# Autodesk Inventor assembly: maze_version2
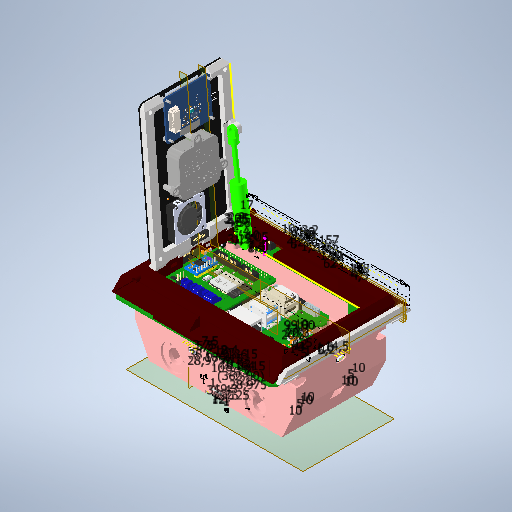
[picture p0: Inventor's stored thumbnail of the model, 512x512]
Saved by Autodesk Inventor 2025 (Build 290162000, 162)
## iProperties
Created: 2026-06-23
Part Number: maze_version2
Document SubType Name: Assembly
Designer: garin
Author: garin
## Documents named in this file (20)
- C:\Users\Leva\Documents\Git\TheseusV2_Maze\Construction\Theseus_v2\Theseus_v2.iam
- C:\Users\Leva\Documents\Git\TheseusV2_Maze\Construction\Theseus_v2\DDSM210.ipt
- C:\Users\Leva\Documents\Git\TheseusV2_Maze\Construction\akkum_TSE\akkum.iam
- C:\Users\Leva\Documents\Git\TheseusV2_Maze\Construction\Theseus_v2\low_part.ipt
- C:\Users\Leva\Documents\Git\TheseusV2_Maze\Construction\Theseus_v2\USBCamera.ipt
- C:\Users\Leva\Documents\Git\TheseusV2_Maze\Construction\maze_test_course\maze_test_course.ipt
- C:\Users\Leva\Documents\Git\TheseusV2_Maze\Construction\Theseus_v2\TCS34725.ipt
- C:\Users\Leva\Documents\Git\TheseusV2_Maze\Construction\Theseus_v2\optopar.ipt
- C:\Users\Leva\Documents\Git\TheseusV2_Maze\Construction\Theseus_v2\magasin.ipt
- C:\Users\Leva\Documents\Git\TheseusV2_Maze\Construction\Theseus_v2\mother_board\mb_mother_board.iam
- C:\Users\Leva\Documents\Git\TheseusV2_Maze\Construction\Theseus_v2\OCS-D008 B.ipt
- C:\Users\Leva\Documents\Git\TheseusV2_Maze\Construction\Theseus_v2\up_part.ipt
- C:\Users\Leva\Documents\Git\TheseusV2_Maze\Construction\Theseus_v2\microswitch_cap.ipt
- C:\Users\Leva\Documents\Git\TheseusV2_Maze\Construction\Theseus_v2\microswitch_cap_MIR.ipt
- C:\Users\Leva\Documents\Git\TheseusV2_Maze\Schematic\TSE_power_control_board\model\TSE_power_control_board.iam
- C:\Users\Leva\Documents\Git\TheseusV2_Maze\Schematic\TSE_sensor_commutation_board\model\TSE_sensor_commutation_board.iam
- C:\Users\Leva\Documents\Git\TheseusV2_Maze\Schematic\TSE_commutation_board\model\TSE_commutation_board.iam
- C:\Users\Leva\Documents\Git\TheseusV2_Maze\Construction\Theseus_v2\cap.ipt
- C:\Users\Leva\Documents\Git\TheseusV2_Maze\Construction\Theseus_v2\gaslift_YQ4-12_body.ipt
- C:\Users\Leva\Documents\Git\TheseusV2_Maze\Construction\Theseus_v2\gaslift_YQ4-12_rod.ipt
## Components (26 placed, 19 different names)
1. low_part:1 — Заподлицо:1, Заподлицо:2, Заподлицо:3, Совмещение:1, Совмещение:2, Совмещение:3, Совмещение:7, Совмещение:8, Совмещение:9, Совмещение:27, Совмещение:28, Совмещение:29, Совмещение:30, Совмещение:31, Совмещение:32, Совмещение:42, Совмещение:43, Совмещение:44, Совмещение:45, Совмещение:46, Совмещение:47, Совмещение:49, Угол:1, Совмещение:62, Совмещение:63, Заподлицо:14, Совмещение:64, Совмещение:65, Заподлицо:18, Совмещение:68, Совмещение:122, Заподлицо:117, Совмещение:123, Совмещение:124, Совмещение:125, Совмещение:129, Заподлицо:118, Заподлицо:119, Заподлицо:122
2. DDSM210:1 — Совмещение:27, Совмещение:28, Совмещение:29, Заподлицо:19
3. DDSM210:2 — Совмещение:1, Совмещение:2, Совмещение:3
4. DDSM210:3 — Совмещение:30, Совмещение:31, Совмещение:32
5. DDSM210:4 — Совмещение:7, Совмещение:8, Совмещение:9
6. akkum:2 [sub-assembly] — Совмещение:122, Заподлицо:117
7. maze_test_course:1 — Совмещение:35
8. TCS34725:1 — Совмещение:45, Совмещение:46, Совмещение:47
9. optopar:1 — Совмещение:42, Совмещение:43, Совмещение:44
10. USBCamera:2 — Совмещение:49, Угол:1, Совмещение:68
11. magasin:1 — Совмещение:62, Совмещение:63, Заподлицо:14, Заподлицо:15
12. mb_mother_board:1 [sub-assembly] — Совмещение:126, Совмещение:127, Совмещение:128
13. OCS-D008 B:1 — Заподлицо:15, Совмещение:64, Совмещение:65
14. up_part:1 — Заподлицо:18, Заподлицо:19, Совмещение:69, Совмещение:70, Совмещение:71, Совмещение:77, Совмещение:78, Совмещение:85, Совмещение:86, Совмещение:88, Совмещение:89, Совмещение:130, Заподлицо:121, Заподлицо:122, Совмещение:131, Совмещение:133, Совмещение:135, Совмещение:137, Совмещение:138
15. USBCamera:3 — Совмещение:69, Совмещение:70, Совмещение:71
16. USBCamera:4
17. microswitch_cap:1 — Совмещение:77, Совмещение:78
18. microswitch_cap_r:1
19. microswitch_cap:2 — Совмещение:88, Совмещение:89
20. microswitch_cap_r:2 — Совмещение:85, Совмещение:86
21. TSE_power_control_board:1 [sub-assembly] — Совмещение:123, Совмещение:124, Совмещение:125, Совмещение:126, Совмещение:127, Совмещение:128
22. TSE_sensor_commutation_board:1 [sub-assembly] — Совмещение:129, Заподлицо:118, Заподлицо:119, Совмещение:130, Заподлицо:121
23. TSE_commutation_board:1 [sub-assembly] — Совмещение:134
24. cap:1 — Совмещение:131, Совмещение:133, Совмещение:134, Совмещение:135, Совмещение:139
25. gaslift_YQ4-12_body:1 — Совмещение:136, Совмещение:137, Совмещение:138
26. gaslift_YQ4-12_rod:1 — Совмещение:136, Совмещение:139
## Relationships (64: Mate 51, Flush 12, Angle 1)
- Заподлицо:1 [Flush]: low_part:1
- Заподлицо:2 [Flush]: low_part:1
- Заподлицо:3 [Flush]: low_part:1
- Совмещение:1 [Mate]: low_part:1 ↔ DDSM210:2
- Совмещение:2 [Mate]: low_part:1 ↔ DDSM210:2
- Совмещение:3 [Mate]: low_part:1 ↔ DDSM210:2
- Совмещение:7 [Mate]: low_part:1 ↔ DDSM210:4
- Совмещение:8 [Mate]: low_part:1 ↔ DDSM210:4
- Совмещение:9 [Mate]: low_part:1 ↔ DDSM210:4
- Совмещение:27 [Mate]: low_part:1 ↔ DDSM210:1
- Совмещение:28 [Mate]: low_part:1 ↔ DDSM210:1
- Совмещение:29 [Mate]: low_part:1 ↔ DDSM210:1
- Совмещение:30 [Mate]: low_part:1 ↔ DDSM210:3
- Совмещение:31 [Mate]: low_part:1 ↔ DDSM210:3
- Совмещение:32 [Mate]: low_part:1 ↔ DDSM210:3
- Совмещение:35 [Mate]: maze_test_course:1
- Совмещение:42 [Mate]: low_part:1 ↔ optopar:1
- Совмещение:43 [Mate]: low_part:1 ↔ optopar:1
- Совмещение:44 [Mate]: low_part:1 ↔ optopar:1
- Совмещение:45 [Mate]: low_part:1 ↔ TCS34725:1
- Совмещение:46 [Mate]: low_part:1 ↔ TCS34725:1
- Совмещение:47 [Mate]: low_part:1 ↔ TCS34725:1
- Совмещение:49 [Mate]: low_part:1 ↔ USBCamera:2
- Угол:1 [Angle] (0 deg): low_part:1 ↔ USBCamera:2
- Совмещение:62 [Mate] (0.2 mm): low_part:1 ↔ magasin:1
- Совмещение:63 [Mate] (0.2 mm): low_part:1 ↔ magasin:1
- Заподлицо:14 [Flush] (1.4 mm): low_part:1 ↔ magasin:1
- Заподлицо:15 [Flush] (-0.4 mm): magasin:1 ↔ OCS-D008 B:1
- Совмещение:64 [Mate] (0.5 mm): low_part:1 ↔ OCS-D008 B:1
- Совмещение:65 [Mate] (0.5 mm): low_part:1 ↔ OCS-D008 B:1
- Заподлицо:18 [Flush]: low_part:1 ↔ up_part:1
- Заподлицо:19 [Flush]: DDSM210:1 ↔ up_part:1
- Совмещение:68 [Mate]: low_part:1 ↔ USBCamera:2
- Совмещение:69 [Mate]: up_part:1 ↔ USBCamera:3
- Совмещение:70 [Mate] (0.5 mm): up_part:1 ↔ USBCamera:3
- Совмещение:71 [Mate] (0.5 mm): up_part:1 ↔ USBCamera:3
- Совмещение:77 [Mate] (0.25 mm): up_part:1 ↔ microswitch_cap:1
- Совмещение:78 [Mate] (0.2 mm): up_part:1 ↔ microswitch_cap:1
- Совмещение:85 [Mate] (0.25 mm): up_part:1 ↔ microswitch_cap_r:2
- Совмещение:86 [Mate] (0.2 mm): up_part:1 ↔ microswitch_cap_r:2
- Совмещение:88 [Mate] (0.25 mm): up_part:1 ↔ microswitch_cap:2
- Совмещение:89 [Mate] (0.2 mm): up_part:1 ↔ microswitch_cap:2
- Совмещение:122 [Mate]: low_part:1 ↔ akkum:2
- Заподлицо:117 [Flush]: low_part:1 ↔ akkum:2
- Совмещение:123 [Mate]: low_part:1 ↔ TSE_power_control_board:1
- Совмещение:124 [Mate]: low_part:1 ↔ TSE_power_control_board:1
- Совмещение:125 [Mate]: low_part:1 ↔ TSE_power_control_board:1
- Совмещение:126 [Mate] (2.5 mm): mb_mother_board:1 ↔ TSE_power_control_board:1
- Совмещение:127 [Mate]: mb_mother_board:1 ↔ TSE_power_control_board:1
- Совмещение:128 [Mate]: mb_mother_board:1 ↔ TSE_power_control_board:1
- Совмещение:129 [Mate]: low_part:1 ↔ TSE_sensor_commutation_board:1
- Заподлицо:118 [Flush]: low_part:1 ↔ TSE_sensor_commutation_board:1
- Заподлицо:119 [Flush]: low_part:1 ↔ TSE_sensor_commutation_board:1
- Совмещение:130 [Mate]: up_part:1 ↔ TSE_sensor_commutation_board:1
- Заподлицо:121 [Flush]: up_part:1 ↔ TSE_sensor_commutation_board:1
- Заподлицо:122 [Flush]: low_part:1 ↔ up_part:1
- Совмещение:131 [Mate] (1.1 mm): up_part:1 ↔ cap:1
- Совмещение:133 [Mate]: up_part:1 ↔ cap:1
- Совмещение:134 [Mate]: TSE_commutation_board:1 ↔ cap:1
- Совмещение:135 [Mate] (1.1 mm): up_part:1 ↔ cap:1
- Совмещение:136 [Mate]: gaslift_YQ4-12_body:1 ↔ gaslift_YQ4-12_rod:1
- Совмещение:137 [Mate]: up_part:1 ↔ gaslift_YQ4-12_body:1
- Совмещение:138 [Mate]: up_part:1 ↔ gaslift_YQ4-12_body:1
- Совмещение:139 [Mate]: cap:1 ↔ gaslift_YQ4-12_rod:1
